# Autodesk Inventor assembly: FO-021-NT
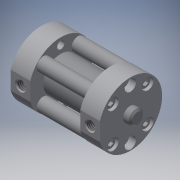
[picture p0: Inventor's stored thumbnail of the model, 180x180]
Saved by Autodesk Inventor 2019.4 (Build 234330000, 330)
## iProperties
Category: PARTsolutions
Company: BIMBA
Created: 2020-02-04
Part Number: FO-021-NT
Catalog Web Link: www.cadenas.de
Description: FO, FOD, FOR, FOS-Bimba FLAT-1
Vendor: BIMBA
Document SubType Name: Assembly
Designer: psadmin
Manufacturer: BIMBA
Mass: 13.508 g
Surface Area: 133.724 cm^2
Volume: 13.508 cm^3
Density: 1 g/cm^3
PSOL_IDENT_0: {$CADENAS_DATA\23d-libs\bimba\bimba_brand\bimba_imperial\bimba_full_line\flat_cylinders\fo1\bif_asmt
PSOL_IDENT_1: ab.prj},318 {VTYP=3D},{STYP=ASSTAB},{NB=FO-021-NT},{LINA=FO-021-NT},{NN=FO, FOD, FOR, FOS},{DATE=22.
PSOL_IDENT_2: 01.2020 09:06:06},{GEOMDATE=12.06.2019 07:36:45},{VERSION=},{LINEID=10},{WBVAR=STROKE,ACTING,MNTR,MN
PSOL_IDENT_3: TF,EE,EEL,TWAB,B,RT,LPHD,G,HR,FO,CRB,FS,M,PP,TO,RM,UM,STPT1,STPT3,STPT4,STPTU1,STPTU3,STPTU4,MRS,W,C
PSOL_IDENT_4: B,TB},{WBNUMERIC=STROKE,EEL}  {NB=FO-021-NT},{LINA=FO-021-NT},{KT=DUMMY},{PN=FO-021-NT},{PNA=(NO ACC
PSOL_IDENT_5: ESSORIES)},{PNC=FO-021-NT},{BORE=9/16\" (02)},{BORE1=0.56250000},{BOREPN=02},{STROKE=1},{STROKEMIN=0
PSOL_IDENT_6: .12500},{STROKEMAX=16.00000000},{ACTING=},{ACTINGALG='','Double Acting, Single End Rod [FO]', 'D'  ,
PSOL_IDENT_7: 'Double Acting, Double End Rod [FOD]', 'R', 'Reverse Acting [FOR]', 'S'  ,'Single Acting [FOS]'},{M
PSOL_IDENT_8: NTR=},{MNTF=},{MNT=},{MNTALG='','Standard Counterbored Mounting Holes','1','Pivot Mount','1N','Pivot
PSOL_IDENT_9: Mount 90 Deg. from Standard','3','Threaded Mounting Holes, Both Ends','3F','Threaded Mounting Holes
PSOL_IDENT_10: , Front','3R','Threaded Mounting Holes, Rear','4','Screw Clearance Holes, Both Ends','4F','Screw Cle
PSOL_IDENT_11: arance Holes, Front','4R','Screw Clearance Holes, Rear','5','Nose Mount'},{EEMAX=17},{EE=},{EEALG=''
PSOL_IDENT_12: ,'Without Extra Extension','EE','With Extra Extension'},{EEL=0.000},{EELALG=0},{OPLALG='','Standard
PSOL_IDENT_13: Grease Lube','99','Oil Pre-Lube [99]'},{TWAB=},{TWABALG='','Standard Stainless Steel Body' },{B=},{B
PSOL_IDENT_14: ALG='','Without Bumper','B','Bumper, Both Ends','BR','Bumper, Rear Only','BF','Bumper, Front Only'},
PSOL_IDENT_15: {RT=NT},{RTALG='', 'Standard Female Thread #8-32 UNC-2B', 'MT', 'Male Rod End (Fine) #8-32 UNC-2B [M
PSOL_IDENT_16: T]', 'NT'  , 'Non-Threaded Rod (Plain Rod) [NT]'},{LPHD=},{LPHDALG='','Standard Pressure Design','D'
PSOL_IDENT_17: ,'Low Pressure Hydraulic Design (250 psi max) [D]'},{G=},{GALG='','Standard Grease Lube','99','Oil P
PSOL_IDENT_18: re-Lube [99]'},{HR=},{HRALG='','N/A'},{HD=},{HDALG='', 'N/A'},{FO=},{FOALG='','N/A'},{CRB=},{CRBALG=''
PSOL_IDENT_19: ,'Standard Rod Bushing','K','Composite Rod Bushing [K]'},{FS=},{FSALG='','Standard Friction Seals','
PSOL_IDENT_20: L','Low Friction Seals', 'X', 'Ring Rod Seal'},{FSPNL=},{FSPNX=},{M=},{MALG='','Without Magnetic Pos
PSOL_IDENT_21: ition Sensing','M','With Magnetic Position Sensing [M]','M1','With Magnetic Position Sensing (Positi
PSOL_IDENT_22: on 1) [M1]','M3','With Magnetic Position Sensing (Position 3) [M3]' ,'M4','With Magnetic Position Se
PSOL_IDENT_23: nsing (Position 4) [M4]' },{PB=},{PBALG='','Standard Body','PB','Composite Body [PB]'},{PP=},{PPALG=''
PSOL_IDENT_24: ,'Standard (ports in line, position #1)'},{TO=},{TOALG= '', 'Standard Temp', 'Q'  , 'Low Temperature
PSOL_IDENT_25: Operation (-40°F to 200°F)', 'V'  , 'High Temperature Option (0°F to 400°F)' },{S=},{SALG='','N/A'}
PSOL_IDENT_26: ,{ST=},{STALG= '' , 'N/A' },{RM=},{RMALG='', 'Chrome Plated Stainless Steel', 'SR'  , 'Non-Chrome Pl
PSOL_IDENT_27: ated Stainless Steel Rod [SR]'},{UM=},{STPT1=},{STPT1ALG= '' , 'N/A' },{STPT2=},{STPT2ALG= '' , 'N/A'
PSOL_IDENT_28: },{STPT3=},{STPT3ALG= '' , 'N/A' },{STPT4=},{STPT4ALG= '' , 'N/A' },{UMALG= '','Without Magnetic Po
PSOL_IDENT_29: sition Sensing 90°','U','With Magnetic Position Sensing 90° [U]'  ,'U4','With Magnetic Position Sens
PSOL_IDENT_30: ing 90° (Position 4) [U4]' },{STPTU1=},{STPTU1ALG= '' , 'N/A' },{STPTU3=},{STPTU3ALG= '' , 'N/A' },{
PSOL_IDENT_31: STPTU4=},{STPTU4ALG= '' , 'N/A' },{U4ALG= ,'U4','With Magnetic Position Sensing 90° (Position 4) [U4
PSOL_IDENT_32: ]' },{SOALG='', 'Without Ring Rod Seal', 'X', 'With Ring Rod Seal'},{SO=},{MRS=},{MRSALG='','None ','
PSOL_IDENT_33: Z','Metallic Rod Scraper [Z]'},{W=},{WALG='', 'Without Wiper', 'W', 'With Wiper'},{Y=},{YALG='','N/A'
PSOL_IDENT_34: },{RP=},{CB=},{TB=},{A=1.12},{B1=0.13},{BA=0.56},{BA1=0.56},{BB=0.00},{BB1=0.69},{BC=0.00},{BD=0.00}
PSOL_IDENT_35: ,{B11=-},{C=0.88},{DD=2},{D=#4},{CPIL=0.12000000},{DC=0.18800000},{DCP=0.12000000},{DCD=0.85500000},
PSOL_IDENT_36: {ES=#8-32 UNC-2B},{EC=N/A},{ED=0.460},{F=0.25},{G1=0.14},{H=0.22},{HH=},{J=0.34},{K=0.17},{K1=0.17},
PSOL_IDENT_37: {K2=0.27},{L=#10-32},{ANGLE=45},{LDP=0.20000000},{LP=0.16000000},{LPDP=0.28000000},{TD=0.65700000},{
PSOL_IDENT_38: TDDP=0.10000},{TD1=0.59500},{TD2=0.61000},{TDIN=0.56200},{LSF=0.31250000},{LSFDP=0.02000000},{BC1=0.
PSOL_IDENT_39: 81000},{BC2=1.38000},{BC3=1.96000},{BC4=2.52000},{BD1=1.06000},{BD2=1.62000},{BD3=2.14000},{BD4=2.70
PSOL_IDENT_40: 000},{BBB=0.56},{FSADD1=0.25000000},{HDADD1=0.13000000},{MADD1=0.875},{M1=0.87500000},{M2=0.62500000
PSOL_IDENT_41: },{M3=0.37500000},{RL=1.45},{BL=1.08},{LR=0.88},{FSADD=0},{HDADD=0},{MADD=0},{ER=},{RL22=0.13},{RL11=
PSOL_IDENT_42: 0.13000000},{RL1=0.13},{MNTRG=},{MNTRH=},{LG1=0.38000000},{LG=0},{RPART=0.08},{AA1=0.06},{AB1=0.75},
PSOL_IDENT_43: {AC1=0.38000000},{AD1=1/2-20 UNF-2A},{AE1=0.498},{AF1=0.31},{MM1=N/A},{MM=-},{MM2=0.13},{N=-},{N1=N/
PSOL_IDENT_44: A},{NN=0.24},{P1=0.000},{NB1=0.00000000},{P=-},{R=-},{R1=#4-40 UNC-2B},{R7=#6-32 UNC-2B},{Q=-},{Q1=0
PSOL_IDENT_45: .19},{S1=-},{S2=0.38},{T=-},{T1=0.19},{U=-},{U1=0.25},{W1=-},{W11=0.75},{X=-},{Y1=-},{Z=-},{AA=-},{A
PSOL_IDENT_46: B=-},{AC2=0.00},{AC=-},{AD=-},{AE=-},{AF=-},{Z1=0.19},{Y11=0.63},{X1=0.17},{DASH=-},{RTPN1=},{RTPN2=
PSOL_IDENT_47: NT},{QPN1=},{QPN2=},{EELPN=},{CBALG='','N/A'},{TBALG='','N/A'},{RPALG='','N/A'},{CBPN=},{TBPN=},{RPP
PSOL_IDENT_48: N=},{STPT1PN=},{STPT2PN=},{STPT3PN=},{STPT4PN=},{RPALG1='','N/A'},{CBALG1='','N/A'},{TBALG1='','N/A'
PSOL_IDENT_49: },{CBPN1=},{TBPN1=},{RPPN1=},{CB1=BC-1},{TB1=-},{RP1=RP-1/2},{LR1=0.88},{PPATH=fo1_asmtpl.prj},{MNTR
PSOL_IDENT_50: ALG='','Standard Counterbored Mounting Holes'  ,'1','Pivot Mount','1N','Pivot Mount 90 Deg. from Sta
PSOL_IDENT_51: ndard'   ,'3R','Threaded Mounting Holes, Rear','4R','Screw Clearance Holes, Rear','6','F Series Inte
PSOL_IDENT_52: rchange, Counterbored, Rear [6]' ,'7R','F Series Interchange, Threaded, Rear [7R]'},{MNT2R=},{MNTFAL
PSOL_IDENT_53: G= '','Standard Counterbored Mounting Holes'       ,'3F','Threaded Mounting Holes, Front','4F','Scre
PSOL_IDENT_54: w Clearance Holes, Front'    ,'5','Nose Mount'      ,'7F','F Series Interchange, Threaded, Front [7F
PSOL_IDENT_55: ]'  },{MNT2F=},{MNT5F= ,'5','Nose Mount'  },{MNTPN=},{MNTPNRH=0},{MNTPNRG=0},{WPN=},{HDPN=},{ASSOPTA
PSOL_IDENT_56: CC=W},{MATALGHTML=<b>Flat 1 Cylinders:</b><dl><dt>End Caps & Posts:</dt><dd>- Anodized Aluminum</dd>
PSOL_IDENT_57: <dt> Seals:</dt><dd>- Buna N </dd><dt>Body:</dt><dd>- 304 Stainless Steel</dd><dt>Bearings:</dt><dd>
PSOL_IDENT_58: - Oil Impregnated Bronze</dd><dt>Rod:</dt><dd>-  303 Stainless Steel</dd></dl>},{STRK2D=0},{X2D=2},{
PSOL_IDENT_59: STROKESW=1.000},{EESW=0.000},{FCD=0},{BCD=0},{RCD=0},{CUSTADD=0.0000},{STPTU1PN=},{STPTU3PN=},{STPTU
PSOL_IDENT_60: 4PN=},{FOADD=0.000},{NPTF=NT},{OPLPN=},{GPN=},{TU2CFG=},{TU3CFG=},{TU4CFG=},{MNT4F=,'4F','Screw Clea
PSOL_IDENT_61: rance Holes, Front'},{NPT=-},{HHFT=0.12},{HHCF=N/A},{HHMT=N/A},{HHMTH=N/A},{HHNPT=N/A},{FTL1=0.460},
PSOL_IDENT_62: {NEWPRA=1}
NN: 0.24
NT: Bimba FLAT-1
NB: FO-021-NT
NBSYN: $PNC.
LINA: FO-021-NT
PN: FO-021-NT
PNA: (NO ACCESSORIES)
BORE: 9/16" (02)
STROKE: 1
ACTING: Double Acting, Single End Rod [FO]
MNTR: Standard Counterbored Mounting Holes
MNTF: Standard Counterbored Mounting Holes
EE: Standard Rod Extension
EEL: 0
TWAB: Standard Stainless Steel Body
B: Without Bumper
RT: Non-Threaded Rod (Plain Rod) [NT]
LPHD: Standard Pressure Design
G: Standard Grease Lube
HR: N/A
FO: N/A
CRB: Standard Rod Bushing
FS: Standard O-Ring Seals
M: Without Magnetic Position Sensing
PP: Standard (ports in line, position #1)
TO: Standard -20° to 200°F (-29° to 95°C)
RM: Chrome Plated Stainless Steel
UM: Without Magnetic Position Sensing 90°
STPT1: N/A
STPT3: N/A
STPT4: N/A
STPTU1: N/A
STPTU3: N/A
STPTU4: N/A
W: Without Wiper
CB: N/A
TB: N/A
A: 1.12
B1: 0.13
BA: 0.56
BB: 0
BC: 0
BD: 0
B11: -
C: 0.88
DD: 2
D: #4
ES: #8-32 UNC-2B
EC: N/A
ED: 0.46
F: 0.25
G1: 0.14
H: 0.22
J: 0.34
K: 0.17
L: #10-32
MM: -
MM2: 0.13
N: -
P: -
R: -
Q: -
S1: -
T: -
U: -
W1: -
X: -
Y1: -
Z: -
AA: -
AB: -
AC: -
AD: -
AE: -
AF: -
SUPPLIER: BIMBA
ARTICLENO: FO-021-NT
BOMINFO: FO-021-NT
CREATOR: CADENAS GmbH
Title: FO-021-NT
Author: Cadenas PARTsolutions
Comments: Bimba FLAT-1
## Documents named in this file (8)
- T:\EIT\2020 Infinite Recharge\2020 ROBOT\COMMON PARTS\AIR CYLINDERS\FO-021-NT\AIS2018\FO-021-NT.iam
- T:\EIT\2020 Infinite Recharge\2020 ROBOT\COMMON PARTS\AIR CYLINDERS\FO-021-NT\AIS2018\02-2-0_125-FO1_BM_heads_left-bif.ipt
- T:\EIT\2020 Infinite Recharge\2020 ROBOT\COMMON PARTS\AIR CYLINDERS\FO-021-NT\AIS2018\021_075-FO1_BM_tube.ipt
- T:\EIT\2020 Infinite Recharge\2020 ROBOT\COMMON PARTS\AIR CYLINDERS\FO-021-NT\AIS2018\02-1NT-0_125-FO1_BM_heads-bif.ipt
- T:\EIT\2020 Infinite Recharge\2020 ROBOT\COMMON PARTS\AIR CYLINDERS\FO-021-NT\AIS2018\D-D0144-SS-1_25-bif.ipt
- T:\EIT\2020 Infinite Recharge\2020 ROBOT\COMMON PARTS\AIR CYLINDERS\FO-021-NT\AIS2018\POST0_5625-0_875-bif.ipt
- T:\EIT\2020 Infinite Recharge\2020 ROBOT\COMMON PARTS\AIR CYLINDERS\FO-021-NT\AIS2018\FO-0211_444NT-00_rod-bif.ipt
- T:\EIT\2020 Infinite Recharge\2020 ROBOT\COMMON PARTS\AIR CYLINDERS\FO-021-NT\AIS2018\0_56250_075-rod_part0.ipt
## Components (13 placed, 7 different names)
1. 02-2-0_125-FO1_BM_heads_left-bif:1
2. 021_075-FO1_BM_tube:1
3. 02-1NT-0_125-FO1_BM_heads-bif:1 — Insert:2
4. D-D0144-SS-1_25-bif:1
5. D-D0144-SS-1_25-bif:2
6. D-D0144-SS-1_25-bif:3
7. D-D0144-SS-1_25-bif:4
8. POST0_5625-0_875-bif:1
9. POST0_5625-0_875-bif:2
10. POST0_5625-0_875-bif:3
11. POST0_5625-0_875-bif:4
12. FO-0211_444NT-00_rod-bif:1 — Insert:1
13. 0_56250_075-rod_part0:1 — Insert:1, Insert:2
## Relationships (2: Insert 2)
- Insert:1: FO-0211_444NT-00_rod-bif:1 ↔ 0_56250_075-rod_part0:1
- Insert:2: 02-1NT-0_125-FO1_BM_heads-bif:1 ↔ 0_56250_075-rod_part0:1
